# Autodesk Inventor assembly: Assembly1
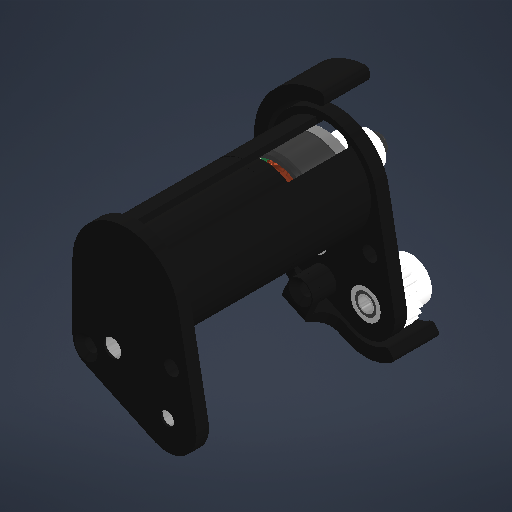
[picture p0: Inventor's stored thumbnail of the model, 512x512]
Saved by Autodesk Inventor 2026.1 (Build 301233020, 233B)
## iProperties
Created: 2026-04-15
Part Number: Assembly1
Document SubType Name: Assembly
Designer: Bahaa
Mass: 42.2903 g
Surface Area: 220.638 cm^2
Volume: 25.0632 cm^3
Density: 1.68734 g/cm^3
Author: Bahaa
## Documents named in this file (10)
- C:\Users\Bahaa\Nextcloud2\CAD\25-26\V2\Dribbler\Dribbler.iam
- C:\Users\Bahaa\Nextcloud2\CAD\25-26\V2\Dribbler\Dribbler Bracket A.ipt
- C:\Users\Bahaa\Nextcloud2\CAD\25-26\V2\Dribbler\t-motor-f1507-1.snapshot.1\T-Motor F1507\T-Motor F1507\T-Motor F1507.iam
- C:\Users\Bahaa\Nextcloud2\CAD\25-26\V2\Dribbler\MAEDLER_29102000\29102000.ipt
- C:\Users\Bahaa\Nextcloud2\CAD\25-26\V2\Dribbler\MAEDLER_29102500\29102500.ipt
- C:\Users\Bahaa\Nextcloud2\CAD\25-26\V2\Dribbler\MAEDLER_29103600\29103600.ipt
- C:\Users\Bahaa\Downloads\Dribbler Cover.ipt
- C:\Users\Bahaa\Nextcloud2\CAD\25-26\V2\Dribbler\Dribbler Bracket B.ipt
- C:\Users\Bahaa\Nextcloud2\CAD\25-26\V2\Dribbler\Miniatur Flanschkugellager MF 74 ZZ.ipt
- C:\Users\Bahaa\Nextcloud2\CAD\25-26\V2\Dribbler\Miniatur Flanschkugellager MF 63 2RS.ipt
## Components (11 placed, 9 different names)
1. Dribbler Bracket A:1 — Mate:1, Mate:2, Mate:3, Mate:4, Mate:5, Mate:7, Mate:8, Flush:1, Flush:2, Mate:9, Mate:10, Mate:11, Mate:12, Mate:13, Mate:14, Mate:15, Mate:16, Mate:19, Mate:20
2. T-Motor F1507:1 [sub-assembly] — Mate:1, Mate:2, Mate:6
3. 29103600:1 — Mate:5, Mate:7
4. 29102500:1 — Mate:4, Mate:8
5. 29102000:1 — Mate:3, Mate:6
6. Dribbler Cover:1 — Flush:1, Flush:2, Mate:9, Mate:10, Mate:11
7. Dribbler Bracket B:1 — Mate:12, Mate:13, Mate:14, Mate:17, Mate:18, Mate:21, Mate:22
8. Miniatur Flanschkugellager MF 74 ZZ:2 — Mate:15, Mate:16
9. Miniatur Flanschkugellager MF 74 ZZ:3 — Mate:17, Mate:18
10. Miniatur Flanschkugellager MF 63 2RS:1 — Mate:19, Mate:20
11. Miniatur Flanschkugellager MF 63 2RS:2 — Mate:21, Mate:22
## Relationships (24: Mate 22, Flush 2)
- Mate:1: Dribbler Bracket A:1 ↔ T-Motor F1507:1
- Mate:2: Dribbler Bracket A:1 ↔ T-Motor F1507:1
- Mate:3: Dribbler Bracket A:1 ↔ 29102000:1
- Mate:4: Dribbler Bracket A:1 ↔ 29102500:1
- Mate:5: Dribbler Bracket A:1 ↔ 29103600:1
- Mate:6: T-Motor F1507:1 ↔ 29102000:1
- Mate:7: Dribbler Bracket A:1 ↔ 29103600:1
- Mate:8: Dribbler Bracket A:1 ↔ 29102500:1
- Flush:1: Dribbler Bracket A:1 ↔ Dribbler Cover:1
- Flush:2: Dribbler Bracket A:1 ↔ Dribbler Cover:1
- Mate:9: Dribbler Bracket A:1 ↔ Dribbler Cover:1
- Mate:10: Dribbler Bracket A:1 ↔ Dribbler Cover:1
- Mate:11: Dribbler Bracket A:1 ↔ Dribbler Cover:1
- Mate:12: Dribbler Bracket A:1 ↔ Dribbler Bracket B:1
- Mate:13: Dribbler Bracket A:1 ↔ Dribbler Bracket B:1
- Mate:14: Dribbler Bracket A:1 ↔ Dribbler Bracket B:1
- Mate:15: Dribbler Bracket A:1 ↔ Miniatur Flanschkugellager MF 74 ZZ:2
- Mate:16: Dribbler Bracket A:1 ↔ Miniatur Flanschkugellager MF 74 ZZ:2
- Mate:17: Dribbler Bracket B:1 ↔ Miniatur Flanschkugellager MF 74 ZZ:3
- Mate:18: Dribbler Bracket B:1 ↔ Miniatur Flanschkugellager MF 74 ZZ:3
- Mate:19: Dribbler Bracket A:1 ↔ Miniatur Flanschkugellager MF 63 2RS:1
- Mate:20: Dribbler Bracket A:1 ↔ Miniatur Flanschkugellager MF 63 2RS:1
- Mate:21: Dribbler Bracket B:1 ↔ Miniatur Flanschkugellager MF 63 2RS:2
- Mate:22: Dribbler Bracket B:1 ↔ Miniatur Flanschkugellager MF 63 2RS:2
